# Autodesk Inventor assembly: Perry_Assembly
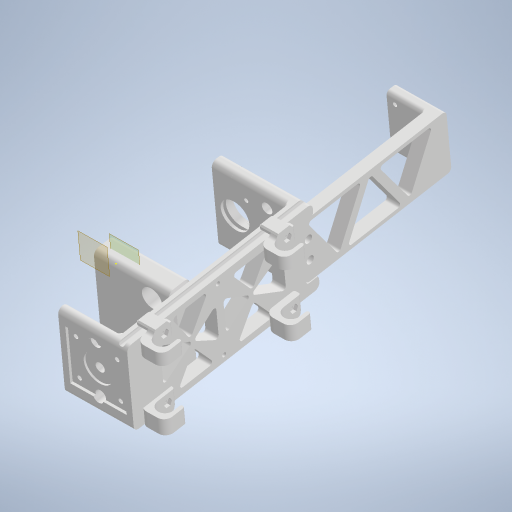
[picture p0: Inventor's stored thumbnail of the model, 512x512]
Saved by Autodesk Inventor 2023 (Build 270158000, 158)
## iProperties
Created: 2023-09-28
Part Number: Perry_Assembly
Document SubType Name: Assembly
Designer: au323799
Author: au323799
## Documents named in this file (8)
- C:\Users\au323799\OneDrive - Aarhus Universitet\A_Articles\ASM_PerryPump\CAD\Perry_Assembly.iam
- C:\Users\au323799\OneDrive - Aarhus Universitet\A_Articles\ASM_PerryPump\CAD\Perry_valve_fixture.ipt
- C:\Users\au323799\OneDrive - Aarhus Universitet\A_Articles\ASM_AuNP\3-Automation\Figures\CAD\Perry_syringe_pump_body.ipt
- C:\Users\au323799\OneDrive - Aarhus Universitet\A_Articles\ASM_AuNP\3-Automation\Figures\CAD\Perry_syringe_pump_sledge.ipt
- C:\Users\au323799\OneDrive - Aarhus Universitet\A_Articles\ASM_PerryPump\CAD\Perry_syringe_fitter_20mL.ipt
- C:\Users\au323799\OneDrive - Aarhus Universitet\A_Articles\ASM_PerryPump\CAD\Perry_plunge_fitter_20ml.ipt
- C:\Users\au323799\OneDrive - Aarhus Universitet\A_Articles\ASM_PerryPump\CAD\Perry_hanger_right.ipt
- C:\Users\au323799\OneDrive - Aarhus Universitet\A_Articles\ASM_PerryPump\CAD\Perry_hanger_left.ipt
## Components (9 placed, 7 different names)
1. Perry_valve_fixture:1 — Rigid:1
2. Perry_syringe_pump_body:1 — Rigid:1, Flush:2, Mate:4, Mate:5, Mate:6, Rotational:1, Mate:7, Mate:8, Rotational:2, Mate:9, Cylindrical:1, Rotational:3, Mate:10, Mate:11, Mate:12, Flush:3
3. Perry_syringe_pump_sledge:1 — Mate:1, Mate:2, Flush:1, Flush:2
4. Perry_plunge_fitter_20ml:1 — Mate:1, Mate:2, Flush:1
5. Perry_syringe_fitter_20mL:1 — Mate:4, Mate:12, Flush:3
6. Perry_hanger_right:1 — Mate:5, Mate:8, Rotational:2
7. Perry_hanger_right:2 — Mate:6, Rotational:1, Mate:7
8. Perry_hanger_left:1 — Cylindrical:1, Mate:11
9. Perry_hanger_left:2 — Mate:9, Rotational:3, Mate:10
## Relationships (19: Mate 11, Flush 3, RevoluteJoint 3, WeldJoint 1, CylindricalJoint 1)
- Rigid:1 [WeldJoint]: Perry_valve_fixture:1 ↔ Perry_syringe_pump_body:1
- Mate:1: Perry_syringe_pump_sledge:1 ↔ Perry_plunge_fitter_20ml:1
- Mate:2: Perry_syringe_pump_sledge:1 ↔ Perry_plunge_fitter_20ml:1
- Flush:1: Perry_syringe_pump_sledge:1 ↔ Perry_plunge_fitter_20ml:1
- Flush:2: Perry_syringe_pump_body:1 ↔ Perry_syringe_pump_sledge:1
- Mate:4: Perry_syringe_pump_body:1 ↔ Perry_syringe_fitter_20mL:1
- Mate:5: Perry_syringe_pump_body:1 ↔ Perry_hanger_right:1
- Mate:6: Perry_syringe_pump_body:1 ↔ Perry_hanger_right:2
- Rotational:1 [RevoluteJoint]: Perry_syringe_pump_body:1 ↔ Perry_hanger_right:2
- Mate:7: Perry_syringe_pump_body:1 ↔ Perry_hanger_right:2
- Mate:8: Perry_syringe_pump_body:1 ↔ Perry_hanger_right:1
- Rotational:2 [RevoluteJoint]: Perry_syringe_pump_body:1 ↔ Perry_hanger_right:1
- Mate:9: Perry_syringe_pump_body:1 ↔ Perry_hanger_left:2
- Cylindrical:1: Perry_syringe_pump_body:1 ↔ Perry_hanger_left:1
- Rotational:3 [RevoluteJoint]: Perry_syringe_pump_body:1 ↔ Perry_hanger_left:2
- Mate:10: Perry_syringe_pump_body:1 ↔ Perry_hanger_left:2
- Mate:11: Perry_syringe_pump_body:1 ↔ Perry_hanger_left:1
- Mate:12: Perry_syringe_pump_body:1 ↔ Perry_syringe_fitter_20mL:1
- Flush:3: Perry_syringe_pump_body:1 ↔ Perry_syringe_fitter_20mL:1
